# Autodesk Inventor assembly: bevelgear_ass
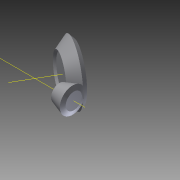
[picture p0: Inventor's stored thumbnail of the model, 180x180]
Saved by Autodesk Inventor 2011 (Build 150239000, 239)
## iProperties
Created: 2005-03-17
Part Number: bevelgear_ass
Document SubType Name: Assembly
Designer: Miroslav Petele
Control State: 0
Master: False
Checked Out: False
Shininess: 64.0
Angle Display Precision: 2
Document Length Units: 11269
Document Angle Units: 11279
Document Time Units: 11290
Document Mass Units: 11283
Document Length Units Precision: 3
Document Angle Units Precision: 2
Density: 0.0
Volumn: 0.0
Area: 0.0
PropertySet Name: Model Information
Author: Miroslav Petele
## Documents named in this file (3)
- C:\Program Files\MITCalc\inventor\bevelgear\bevelgear_ass.iam
- C:\Program Files\MITCalc\inventor\bevelgear\bevelgear_pinion.ipt
- C:\Program Files\MITCalc\inventor\bevelgear\bevelgear_wheel.ipt
## Components (2 placed, 2 different names)
1. bevelgear_pinion:1 — Mate:1, Mate:2
2. bevelgear_wheel:1 — Mate:1, Mate:2
## Relationships (2: Mate 2)
- Mate:1: bevelgear_pinion:1 ↔ bevelgear_wheel:1
- Mate:2: bevelgear_pinion:1 ↔ bevelgear_wheel:1
